# Autodesk Inventor assembly: Automatic plant culture media filling station
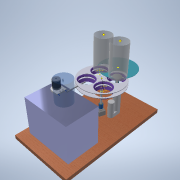
[picture p0: Inventor's stored thumbnail of the model, 180x180]
Saved by Autodesk Inventor 2021.3 (Build 253353010, 353A)
## iProperties
Created: 2015-11-30
Part Number: Automatic plant culture media filling station
Document SubType Name: Assembly
Designer: zwrouse
Author: zwrouse
## Documents named in this file (13)
- C:\Users\Dell\Desktop\Automatic plant culture media filling station.iam
- C:\Users\Dell\Downloads\plate-pouring-system-1.snapshot.9\CAD Files\NEMA Motor 17.ipt
- C:\Users\Dell\Downloads\plate-pouring-system-1.snapshot.9\CAD Files\Shaft Coupling.ipt
- C:\Users\Dell\Downloads\plate-pouring-system-1.snapshot.9\CAD Files\Short Axle.ipt
- C:\Users\Dell\Downloads\plate-pouring-system-1.snapshot.9\CAD Files\Base Stage.ipt
- C:\Users\Dell\Downloads\plate-pouring-system-1.snapshot.9\CAD Files\base plate cone.ipt
- C:\Users\Dell\Downloads\plate-pouring-system-1.snapshot.9\CAD Files\Lid Cone.ipt
- C:\Users\Dell\Downloads\plate-pouring-system-1.snapshot.9\CAD Files\Actuator new.ipt
- C:\Users\Dell\Downloads\plate-pouring-system-1.snapshot.9\CAD Files\actuator.ipt
- C:\Users\Dell\Downloads\Media and indication.iam
- C:\Users\Dell\Downloads\rack holder (2).ipt
- C:\Users\Dell\Downloads\Petriplate holder.ipt
- C:\Users\Dell\Downloads\Pipe.ipt
## Components (20 placed, 12 different names)
1. NEMA Motor 17:1 — Flush:1, Mate:1, Flush:2, Mate:2, Flush:3
2. Shaft Coupling:1 — Flush:2, Mate:2, Rigid:2
3. Short Axle:1 — Rigid:2, Rotational:1
4. Base Stage:1 — Rigid:3, Mate:3, Mate:4, Mate:5, Mate:6
5. Base Stage:2 — Rigid:3, Rotational:1, Rigid:4, Rigid:5, Rigid:6, Rigid:7
6. base plate cone:1 — Mate:4
7. base plate cone:2 — Mate:6
8. base plate cone:3 — Mate:3
9. base plate cone:4 — Mate:5
10. Lid Cone:1 — Rigid:6
11. Lid Cone:2 — Rigid:4
12. Lid Cone:3 — Rigid:7
13. Lid Cone:4 — Rigid:5
14. Actuator new:1 — Cylindrical:1, Flush:3
15. actuator:1 — Cylindrical:1
16. Media and indication:1 [sub-assembly]
17. rack holder (2):1
18. Petriplate holder:1
19. Petriplate holder:2
20. Pipe:1
## Relationships (17: Mate 6, WeldJoint 6, Flush 3, RevoluteJoint 1, CylindricalJoint 1)
- Flush:1: NEMA Motor 17:1
- Mate:1: NEMA Motor 17:1
- Flush:2: NEMA Motor 17:1 ↔ Shaft Coupling:1
- Mate:2: NEMA Motor 17:1 ↔ Shaft Coupling:1
- Rigid:2 [WeldJoint]: Shaft Coupling:1 ↔ Short Axle:1
- Rigid:3 [WeldJoint] (25.4 mm): Base Stage:1 ↔ Base Stage:2
- Rotational:1 [RevoluteJoint]: Short Axle:1 ↔ Base Stage:2
- Mate:3: Base Stage:1 ↔ base plate cone:3
- Mate:4: Base Stage:1 ↔ base plate cone:1
- Mate:5: Base Stage:1 ↔ base plate cone:4
- Mate:6: Base Stage:1 ↔ base plate cone:2
- Rigid:4 [WeldJoint]: Base Stage:2 ↔ Lid Cone:2
- Rigid:5 [WeldJoint]: Base Stage:2 ↔ Lid Cone:4
- Rigid:6 [WeldJoint]: Base Stage:2 ↔ Lid Cone:1
- Rigid:7 [WeldJoint]: Base Stage:2 ↔ Lid Cone:3
- Cylindrical:1: Actuator new:1 ↔ actuator:1
- Flush:3: NEMA Motor 17:1 ↔ Actuator new:1
